# Autodesk Inventor assembly: finalassy
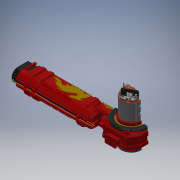
[picture p0: Inventor's stored thumbnail of the model, 180x180]
Saved by Autodesk Inventor 2018 (Build 220112000, 112)
## iProperties
Created: 2019-03-10
Part Number: finalassy
Material: 一般
Document SubType Name: Assembly
Designer: ku_sk
Author: ku_sk
## Documents named in this file (16)
- D:\Inventor\BayBladeLauncher\type2\finalassy.iam
- D:\Inventor\BayBladeLauncher\type2\parts\basecad.ipt
- D:\Inventor\BayBladeLauncher\type2\parts\topcover.ipt
- D:\Inventor\BayBladeLauncher\reedy_540_rc_motor-1.snapshot.2\motor.iam
- D:\Inventor\BayBladeLauncher\type2\parts\bearing.ipt
- D:\Inventor\BayBladeLauncher\type2\parts\frange.ipt
- D:\Inventor\BayBladeLauncher\type2\parts\conectcover.ipt
- D:\Inventor\BayBladeLauncher\type2\parts\conecter.ipt
- D:\Inventor\BayBladeLauncher\type2\parts\switch.ipt
- D:\Inventor\BayBladeLauncher\type2\parts\ring.ipt
- D:\Inventor\BayBladeLauncher\type2\parts\cover.ipt
- D:\Inventor\BayBladeLauncher\type2\parts\bar.ipt
- D:\Inventor\BayBladeLauncher\type2\parts\battery.ipt
- D:\Inventor\BayBladeLauncher\type2\parts\dragon.ipt
- D:\Inventor\BayBladeLauncher\type2\parts\dragon_MIR.ipt
- D:\Inventor\BayBladeLauncher\type2\parts\skyrimlogo2_1_9.ipt
## Components (15 placed, 15 different names)
1. basecad:1 — メイト:1, メイト:2, メイト:3, メイト:4, メイト:5, メイト:6, メイト:10, メイト:11, メイト:14, メイト:15, メイト:16, フラッシュ:1, メイト:22, メイト:23, メイト:29, メイト:30, メイト:31, メイト:32, メイト:33, メイト:34, メイト:35, メイト:36, メイト:37, メイト:38, 角度:1
2. topcover:1 — メイト:4, メイト:5, メイト:6, メイト:7, メイト:9, メイト:24, メイト:25, メイト:26, メイト:27, メイト:28, フラッシュ:3, メイト:39
3. motor:1 [sub-assembly] — メイト:7, メイト:9, メイト:12, メイト:13
4. bearing:1 — メイト:10, メイト:11, メイト:19
5. frange:1 — メイト:12, メイト:13, メイト:20, メイト:21
6. conectcover:1 — メイト:14, メイト:15, メイト:16
7. conecter:1 — メイト:19, フラッシュ:1, フラッシュ:2, メイト:21
8. switch:1 — メイト:22, メイト:23
9. ring:1 — メイト:24, メイト:25, フラッシュ:3
10. cover:1 — メイト:26, メイト:27, メイト:28
11. bar:1 — メイト:29, メイト:30, 角度:1
12. battery:1 — メイト:31, メイト:32
13. dragon:1 — メイト:33, メイト:34, メイト:35
14. dragon_MIR:1 — メイト:36, メイト:37, メイト:38
15. skyrimlogo2_1_9:1 — メイト:39
## Relationships (40: Mate 36, Flush 3, Angle 1)
- メイト:1 [Mate]: basecad:1
- メイト:2 [Mate]: basecad:1
- メイト:3 [Mate]: basecad:1
- メイト:4 [Mate]: basecad:1 ↔ topcover:1
- メイト:5 [Mate]: basecad:1 ↔ topcover:1
- メイト:6 [Mate]: basecad:1 ↔ topcover:1
- メイト:7 [Mate]: topcover:1 ↔ motor:1
- メイト:9 [Mate]: topcover:1 ↔ motor:1
- メイト:10 [Mate]: basecad:1 ↔ bearing:1
- メイト:11 [Mate]: basecad:1 ↔ bearing:1
- メイト:12 [Mate]: motor:1 ↔ frange:1
- メイト:13 [Mate]: motor:1 ↔ frange:1
- メイト:14 [Mate]: basecad:1 ↔ conectcover:1
- メイト:15 [Mate]: basecad:1 ↔ conectcover:1
- メイト:16 [Mate]: basecad:1 ↔ conectcover:1
- メイト:19 [Mate]: bearing:1 ↔ conecter:1
- フラッシュ:1 [Flush] (-12 mm): basecad:1 ↔ conecter:1
- フラッシュ:2 [Flush]: conecter:1
- メイト:20 [Mate]: frange:1
- メイト:21 [Mate]: frange:1 ↔ conecter:1
- メイト:22 [Mate]: basecad:1 ↔ switch:1
- メイト:23 [Mate]: basecad:1 ↔ switch:1
- メイト:24 [Mate]: topcover:1 ↔ ring:1
- メイト:25 [Mate]: topcover:1 ↔ ring:1
- メイト:26 [Mate]: topcover:1 ↔ cover:1
- メイト:27 [Mate]: topcover:1 ↔ cover:1
- メイト:28 [Mate]: topcover:1 ↔ cover:1
- フラッシュ:3 [Flush]: topcover:1 ↔ ring:1
- メイト:29 [Mate]: basecad:1 ↔ bar:1
- メイト:30 [Mate] (1 mm): basecad:1 ↔ bar:1
- メイト:31 [Mate] (0.25 mm): basecad:1 ↔ battery:1
- メイト:32 [Mate]: basecad:1 ↔ battery:1
- メイト:33 [Mate]: basecad:1 ↔ dragon:1
- メイト:34 [Mate]: basecad:1 ↔ dragon:1
- メイト:35 [Mate]: basecad:1 ↔ dragon:1
- メイト:36 [Mate]: basecad:1 ↔ dragon_MIR:1
- メイト:37 [Mate]: basecad:1 ↔ dragon_MIR:1
- メイト:38 [Mate]: basecad:1 ↔ dragon_MIR:1
- メイト:39 [Mate]: topcover:1 ↔ skyrimlogo2_1_9:1
- 角度:1 [Angle] (180 deg): basecad:1 ↔ bar:1
